# Autodesk Inventor assembly: Green HS 84
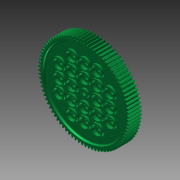
[picture p0: Inventor's stored thumbnail of the model, 180x180]
Saved by Autodesk Inventor 2014 SP1 (Build 180222100, 222)
## iProperties
Created: 2014-02-23
Part Number: Green HS 84
Document SubType Name: Assembly
Designer: Ryan
Author: Ryan
## Documents named in this file (2)
- C:\Users\Ryan\Desktop\sw\lib\Aperture VEX CAD Library\Gears\High Strength Gears\Green HS 84.iam
- C:\Users\Ryan\Desktop\sw\lib\Aperture VEX CAD Library\Gears\High Strength Gears\84-Tooth Gear - no knob.ipt
## Components (2 placed, 1 different names)
1. 84-Tooth Gear - no knob:1 — Mate:1, Mate:2, Mate:3
2. 84-Tooth Gear - no knob:2 — Mate:1, Mate:2, Mate:3
## Relationships (3: Mate 3)
- Mate:1: 84-Tooth Gear - no knob:1 ↔ 84-Tooth Gear - no knob:2
- Mate:2: 84-Tooth Gear - no knob:1 ↔ 84-Tooth Gear - no knob:2
- Mate:3: 84-Tooth Gear - no knob:1 ↔ 84-Tooth Gear - no knob:2
